# Autodesk Inventor assembly: McCrea_koleso_walle_MIR
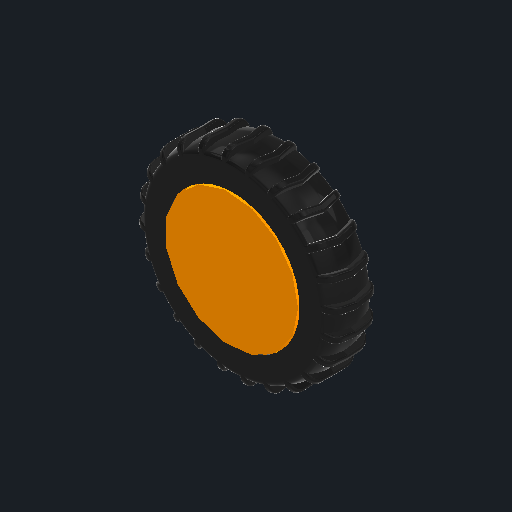
[picture p0: Inventor's stored thumbnail of the model, 512x512]
Saved by Autodesk Inventor 2022 (Build 260153000, 153)
## iProperties
Created: 2022-02-21
Part Number: McCrea_koleso_walle_MIR
Document SubType Name: Assembly
Designer: MatusBarany
Author: MatusBarany
## Documents named in this file (3)
- C:\Users\MatusBarany\Documents\Inventor\wall-e\matus\electronic truck\McCrea_koleso_walle_MIR.iam
- C:\Users\MatusBarany\Documents\Inventor\wall-e\matus\electronic truck\McCrea_guma_walle_MIR.ipt
- C:\Users\MatusBarany\Documents\Inventor\wall-e\matus\electronic truck\McCrea_koleso_jadro_walle_MIR.ipt
## Components (2 placed, 2 different names)
1. McCrea_guma_walle_MIR:1 — Rotational:1
2. McCrea_koleso_jadro_walle_MIR:1 — Rotational:1
## Relationships (1: RevoluteJoint 1)
- Rotational:1 [RevoluteJoint]: McCrea_guma_walle_MIR:1 ↔ McCrea_koleso_jadro_walle_MIR:1
